# Autodesk Inventor assembly: Zespół1
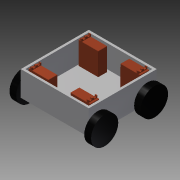
[picture p0: Inventor's stored thumbnail of the model, 180x180]
Saved by Autodesk Inventor 2014 (Build 180170000, 170)
## iProperties
Created: 2013-10-14
Part Number: Zespół1
Document SubType Name: Assembly
Designer: Wojciech
Author: Wojciech
## Documents named in this file (4)
- C:\Users\Wojciech\Desktop\sumo\Zespół1.iam
- C:\Users\Wojciech\Desktop\sumo\korpus.ipt
- C:\Users\Wojciech\Desktop\sumo\koło.ipt
- C:\Users\Wojciech\Desktop\sumo\Serwo.ipt
## Components (9 placed, 3 different names)
1. korpus:1 — Obrotowe:1, Obrotowe:2, Obrotowe:3, Obrotowe:4, Równoległy:1
2. koło:1 — Obrotowe:1, Obrotowe:8
3. koło:2 — Obrotowe:2, Obrotowe:7
4. koło:3 — Obrotowe:3, Obrotowe:5
5. koło:4 — Obrotowe:4, Obrotowe:6
6. Serwo:1 — Obrotowe:8, Równoległy:1
7. Serwo:2 — Obrotowe:7
8. Serwo:3 — Obrotowe:6
9. Serwo:4 — Obrotowe:5
## Relationships (9: RevoluteJoint 8, Flush 1)
- Obrotowe:1 [RevoluteJoint] (-15 mm): korpus:1 ↔ koło:1
- Obrotowe:2 [RevoluteJoint] (-15 mm): korpus:1 ↔ koło:2
- Obrotowe:3 [RevoluteJoint] (5 mm): korpus:1 ↔ koło:3
- Obrotowe:4 [RevoluteJoint]: korpus:1 ↔ koło:4
- Obrotowe:5 [RevoluteJoint] (-15 mm): koło:3 ↔ Serwo:4
- Obrotowe:6 [RevoluteJoint] (-15 mm): koło:4 ↔ Serwo:3
- Obrotowe:7 [RevoluteJoint] (-15 mm): koło:2 ↔ Serwo:2
- Obrotowe:8 [RevoluteJoint] (-15 mm): koło:1 ↔ Serwo:1
- Równoległy:1 [Flush]: korpus:1 ↔ Serwo:1
